# Autodesk Inventor assembly: CA[FD1]
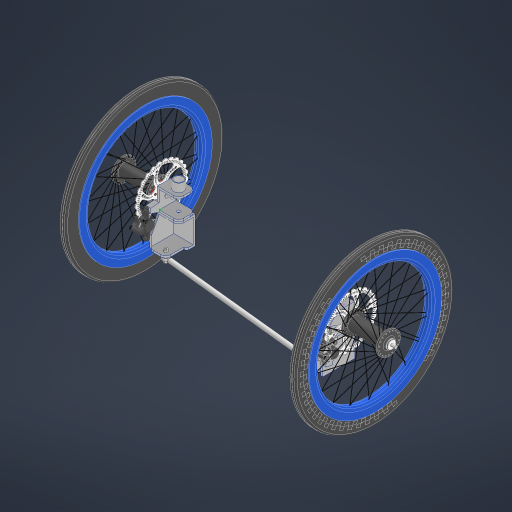
[picture p0: Inventor's stored thumbnail of the model, 512x512]
Saved by Autodesk Inventor 2024 (Build 280153000, 153)
## iProperties
Created: 2023-06-19
Part Number: CA[FD1]
Document SubType Name: Assembly
Designer: juanj
Author: juanj
## Documents named in this file (10)
- C:\Users\juanj\Documents\Documentos\Unisabana\Shell\C23[1stD]\CA[FD1].iam
- C:\Users\juanj\Documents\Documentos\Unisabana\Shell\C23[1stD]\B23[L][FD1].ipt
- C:\Users\juanj\Documents\Documentos\Unisabana\Shell\C23[1stD]\B23[R][FD1].ipt
- C:\Users\juanj\Documents\Documentos\Unisabana\Shell\C23[1stD]\BU23[FD1].ipt
- C:\Users\juanj\Documents\Documentos\Unisabana\Shell\C23[1stD]\C23[L][FD1].ipt
- C:\Users\juanj\Documents\Documentos\Unisabana\Shell\C23[1stD]\C23[R][FD1].ipt
- C:\Users\juanj\Documents\Documentos\Unisabana\Shell\C23[1stD]\DC23[L][FD1].ipt
- C:\Users\juanj\Documents\Documentos\Unisabana\Shell\C23[1stD]\DC23[R][FD1].ipt
- C:\Users\juanj\Documents\Documentos\Unisabana\Shell\C23[1stD]\W23[FD1].ipt
- C:\Users\juanj\Documents\Documentos\Unisabana\Shell\C23[1stD]\D23[FD1].iam
## Components (11 placed, 9 different names)
1. B23[L][FD1]:1 — Insert:8, Angle:4
2. B23[R][FD1]:1 — Insert:9, Angle:5
3. BU23[FD1]:1 — Insert:4, Insert:7
4. C23[L][FD1]:1 — Angle:1, Insert:1, Insert:4, Insert:8
5. C23[R][FD1]:1 — Insert:2, Angle:3, Insert:5, Insert:9
6. DC23[L][FD1]:1 — Angle:1, Insert:1, Angle:2, Insert:3, Flush:1, Angle:4
7. DC23[R][FD1]:1 — Angle:2, Insert:2, Angle:3, Mate:1, Flush:1, Angle:5
8. W23[FD1]:1 — Insert:6
9. BU23[FD1]:2 — Insert:5, Insert:6
10. W23[FD1]:2 — Insert:7
11. D23[FD1]:1 [sub-assembly] — Insert:3, Mate:1
## Relationships (16: Insert 9, Angle 5, Mate 1, Flush 1)
- Angle:1 (0 deg): C23[L][FD1]:1 ↔ DC23[L][FD1]:1
- Insert:1: C23[L][FD1]:1 ↔ DC23[L][FD1]:1
- Angle:2 (0 deg): DC23[L][FD1]:1 ↔ DC23[R][FD1]:1
- Insert:2: C23[R][FD1]:1 ↔ DC23[R][FD1]:1
- Angle:3 (0 deg): C23[R][FD1]:1 ↔ DC23[R][FD1]:1
- Insert:3: DC23[L][FD1]:1 ↔ D23[FD1]:1
- Mate:1: DC23[R][FD1]:1 ↔ D23[FD1]:1
- Flush:1: DC23[L][FD1]:1 ↔ DC23[R][FD1]:1
- Insert:4: BU23[FD1]:1 ↔ C23[L][FD1]:1
- Insert:5: C23[R][FD1]:1 ↔ BU23[FD1]:2
- Insert:6: W23[FD1]:1 ↔ BU23[FD1]:2
- Insert:7: BU23[FD1]:1 ↔ W23[FD1]:2
- Insert:8: B23[L][FD1]:1 ↔ C23[L][FD1]:1
- Angle:4 (0 deg): B23[L][FD1]:1 ↔ DC23[L][FD1]:1
- Insert:9: B23[R][FD1]:1 ↔ C23[R][FD1]:1
- Angle:5 (0 deg): B23[R][FD1]:1 ↔ DC23[R][FD1]:1
